# Autodesk Inventor assembly: preview
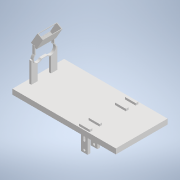
[picture p0: Inventor's stored thumbnail of the model, 180x180]
Saved by Autodesk Inventor 2022 (Build 260153000, 153)
## iProperties
Created: 2022-02-09
Part Number: preview
Document SubType Name: Assembly
Designer: Iñigo
Author: Iñigo
## Documents named in this file (4)
- D:\proyectos\FoBo\model\preview.iam
- D:\proyectos\FoBo\model\main_base.ipt
- D:\proyectos\FoBo\model\motor_fastening.ipt
- D:\proyectos\FoBo\model\ultrasonic_fastening.ipt
## Components (6 placed, 3 different names)
1. main_base:1 — Mate:1, Mate:2, Mate:3, Mate:4, Mate:5, Mate:6, Mate:7, Mate:8, Mate:9, Mate:10, Mate:11, Mate:12, Mate:13
2. motor_fastening:1 — Mate:1, Mate:2, Mate:3
3. motor_fastening:2 — Mate:4, Mate:5, Mate:6
4. motor_fastening:3 — Mate:7, Mate:8, Mate:9
5. motor_fastening:4 — Mate:10, Mate:11, Mate:12
6. ultrasonic_fastening:1 — Mate:13
## Relationships (13: Mate 13)
- Mate:1: main_base:1 ↔ motor_fastening:1
- Mate:2: main_base:1 ↔ motor_fastening:1
- Mate:3: main_base:1 ↔ motor_fastening:1
- Mate:4: main_base:1 ↔ motor_fastening:2
- Mate:5: main_base:1 ↔ motor_fastening:2
- Mate:6: main_base:1 ↔ motor_fastening:2
- Mate:7: main_base:1 ↔ motor_fastening:3
- Mate:8: main_base:1 ↔ motor_fastening:3
- Mate:9: main_base:1 ↔ motor_fastening:3
- Mate:10: main_base:1 ↔ motor_fastening:4
- Mate:11: main_base:1 ↔ motor_fastening:4
- Mate:12: main_base:1 ↔ motor_fastening:4
- Mate:13: main_base:1 ↔ ultrasonic_fastening:1
